# Autodesk Inventor assembly: CL3-100
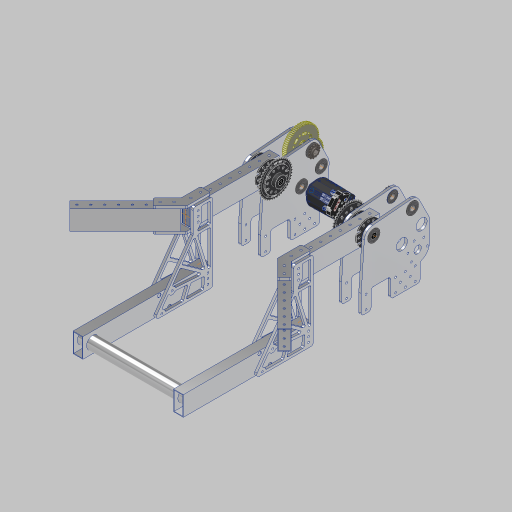
[picture p0: Inventor's stored thumbnail of the model, 512x512]
Saved by Autodesk Inventor 2023.5 (Build 275446000, 446)
## iProperties
Created: 2025-01-28
Part Number: CL3-100
Document SubType Name: Assembly
Designer: slick
Mass: 5966.39 g
Surface Area: 14199.1 cm^2
Volume: 2256.64 cm^3
Density: 2.64392 g/cm^3
Author: slick
## Documents named in this file (22)
- C:\Users\slick\OneDrive\Desktop\2025-ReefScape---CAD\Climber\CL3\CL3-100.iam
- C:\Users\slick\OneDrive\Desktop\2025-ReefScape---CAD\Climber\CL3\CL3-001.ipt
- C:\Users\slick\OneDrive\Desktop\2025-ReefScape---CAD\Climber\CL3\CL3-002.ipt
- C:\Users\slick\OneDrive\Desktop\2025-ReefScape---CAD\Climber\CL3\CL3-003.ipt
- C:\Users\slick\OneDrive\Desktop\2025-ReefScape---CAD\Climber\CL3\CL3-006.ipt
- C:\Users\slick\OneDrive\Desktop\2025-ReefScape---CAD\Field Items\Full Field\FE-2025\GE-25201.iam
- C:\Users\slick\OneDrive\Desktop\2025-ReefScape---CAD\Climber\CL3\CL3-009.ipt
- C:\Users\slick\OneDrive\Desktop\2025-ReefScape---CAD\Elevator\EL2\EL2-005.ipt
- C:\Users\slick\OneDrive\Desktop\2025-ReefScape---CAD\Climber\CL3\CL3-010.ipt
- C:\Users\slick\OneDrive\Desktop\2025-ReefScape---CAD\Climber\CL3\CL3-011.ipt
- C:\Users\slick\OneDrive\Desktop\2025-ReefScape---CAD\COMMON PARTS\HUBS\WCP-1388.ipt
- C:\Users\slick\OneDrive\Desktop\2025-ReefScape---CAD\COMMON PARTS\SPROCKETS\25\WCP-0967 42t 25_chain.ipt
- C:\Users\slick\OneDrive\Desktop\2025-ReefScape---CAD\Climber\CL3\CL3-013.ipt
- C:\Users\slick\OneDrive\Desktop\2025-ReefScape---CAD\Climber\CL3\CL3-014.ipt
- C:\Users\slick\OneDrive\Desktop\2025-ReefScape---CAD\Climber\CL3\CL3-015.ipt
- C:\Users\slick\OneDrive\Desktop\2025-ReefScape---CAD\COMMON PARTS\MOTORS\Kracken with Cover and Boards.iam
- C:\Users\slick\OneDrive\Desktop\2025-ReefScape---CAD\COMMON PARTS\GEARS\WCP-1006\WCP-1006.ipt
- C:\Users\slick\OneDrive\Desktop\2025-ReefScape---CAD\COMMON PARTS\GEARS\20dp .5 hex\72t_Aluminum_Spur_Gear_20_DP_1_2_Hex_Bore_217-3576.ipt
- C:\Users\slick\OneDrive\Desktop\2025-ReefScape---CAD\COMMON PARTS\GEARS\20dp .5 hex\66t_Aluminum_Spur_Gear_20_DP_1_2_Hex_Bore_VersaKeys_217-3223.ipt
- C:\Users\slick\OneDrive\Desktop\2025-ReefScape---CAD\COMMON PARTS\GEARS\20dp .5 hex\20t_Aluminum_Spur_Gear_20_DP_1_2_Hex_Bore_217-2702.ipt
- C:\Users\slick\OneDrive\Desktop\2025-ReefScape---CAD\COMMON PARTS\SPROCKETS\25\14t Steel Double Hub Sprocket (#25 Chain, 12 Hex Bore)\14t Steel Double Hub Sprocket (#25 Chain, 12 Hex Bore).ipt
- C:\Users\slick\OneDrive\Desktop\2025-ReefScape---CAD\COMMON PARTS\BEARINGS\13_75mm_1_2_ThunderHex_ID_x_1_125_OD_x_0_313_WD_Flanged_Bearing_217-4006_MIR.ipt
## Components (58 placed, 21 different names)
1. CL3-001:1 — Flush:24, Insert:5, Insert:6, Insert:7, Insert:11, Insert:12, Insert:13, Insert:14, Mate:43, Mate:44, Mate:51, Mate:52, Mate:53, Mate:54, Mate:55, Angle:4, Insert:43, Insert:44, Mate:90
2. CL3-002:1 — Flush:24, Insert:3, Insert:4, Insert:8
3. CL3-003:1 — Insert:26, Insert:27, Mate:56, Mate:57, Insert:48, Insert:49, Insert:50, Insert:51
4. CL3-001:2 — Insert:18, Insert:19, Insert:20, Insert:21, Insert:24, Insert:25, Insert:41, Mate:65, Insert:42, Mate:66, Mate:67
5. CL3-002:2 — Insert:22, Insert:23
6. CL3-003:2 — Mate:33, Mate:34, Insert:15, Insert:16, Insert:17, Insert:45, Insert:46, Insert:47
7. CL3-015:5 — Mate:41, Flush:31, Flush:32, Angle:4, Symmetry:2, Mate:76, Mate:85, Mate:87, Symmetry:4, Mate:93, Insert:61, Insert:62, Insert:63, Insert:64
8. CL3-015:4 — Mate:68, Flush:33, Symmetry:3, Mate:93, Symmetry:5, Insert:65, Insert:67, Flush:47
9. CL3-006:1 — Tangent:1, Mate:21, Mate:33, Mate:34, Mate:56, Mate:57
10. GE-25201:1 [sub-assembly] — Mate:20, Tangent:1, Mate:21
11. CL3-009:1 — Insert:3, Insert:4, Insert:5, Insert:6
12. CL3-009:2 — Insert:7, Insert:8
13. CL3-013:1 — Insert:43, Insert:44
14. CL3-010:1 — Insert:11, Insert:12, Flush:29
15. CL3-010:2 — Insert:13, Insert:14, Insert:16, Insert:17
16. EL2-005:3 — Insert:15, Insert:45
17. CL3-009:3 — Insert:18, Insert:19
18. CL3-009:4 — Insert:20, Insert:21, Insert:22, Insert:23
19. CL3-010:3 — Insert:25, Flush:29, Flush:30
20. CL3-010:4 — Insert:24, Insert:26, Insert:27, Flush:30
21. CL3-011:1 — Mate:55, Mate:81, Mate:96, Flush:48, Flush:49
22. CL3-015:2 — Mate:41, Flush:31, Flush:32, Symmetry:2, Flush:34, Flush:35, Mate:70, Insert:52, Mate:77, Mate:79, Mate:80, Mate:83, Symmetry:4, Insert:57, Insert:58, Insert:59, Insert:60
23. WCP-1388:1 — Mate:43, Mate:44, Mate:51
24. WCP-1388:2 — Mate:52, Mate:53, Mate:54
25. CL3-015:3 — Mate:68, Flush:33, Flush:34, Flush:35, Symmetry:3, Symmetry:5, Insert:66, Insert:68, Flush:47
26. CL3-011:2 — Mate:67, Mate:88, Mate:95, Flush:50, Flush:51
27. WCP-1388:3 — Insert:41, Mate:65
28. WCP-1388:4 — Insert:42, Mate:66
29. CL3-014:1 — Insert:46
30. CL3-014:2 — Insert:47
31. CL3-014:3 — Insert:50
32. CL3-014:4 — Insert:51
33. EL2-005:4 — Insert:48, Insert:49
34. Kracken with Cover and Boards:1 [sub-assembly] — Mate:70, Insert:52, Mate:72, Mate:73, Mate:79
35. WCP-1006:1 — Mate:72, Mate:73
36. 72t_Aluminum_Spur_Gear_20_DP_1_2_Hex_Bore_217-3576:1 — Mate:80, Mate:83, Mate:84
37. 20t_Aluminum_Spur_Gear_20_DP_1_2_Hex_Bore_217-2702:2 — Mate:84, Flush:39, Mate:85
38. 66t_Aluminum_Spur_Gear_20_DP_1_2_Hex_Bore_VersaKeys_217-3223:1 — Mate:76, Flush:39, Mate:86
39. 20t_Aluminum_Spur_Gear_20_DP_1_2_Hex_Bore_217-2702:1 — Mate:77, Flush:38, Mate:86
40. 66t_Aluminum_Spur_Gear_20_DP_1_2_Hex_Bore_VersaKeys_217-3223:2 — Flush:38
41. WCP-0967 42t 25_chain:3 — Insert:53, Insert:54, Flush:45
42. WCP-1388:5 — Insert:53, Insert:54, Mate:81, Flush:48
43. 14t Steel Double Hub Sprocket (#25 Chain, 12 Hex Bore):1 — Mate:87, Flush:45
44. WCP-0967 42t 25_chain:4 — Flush:46
45. WCP-1388:6 — Mate:88, Flush:50
46. 13_75mm_1_2_ThunderHex_ID_x_1_125_OD_x_0_313_WD_Flanged_Bearing_217-4006_MIR:1 — Insert:68
47. 13_75mm_1_2_ThunderHex_ID_x_1_125_OD_x_0_313_WD_Flanged_Bearing_217-4006_MIR:2 — Insert:67, Mate:95, Flush:51
48. 13_75mm_1_2_ThunderHex_ID_x_1_125_OD_x_0_313_WD_Flanged_Bearing_217-4006_MIR:3 — Insert:65
49. 13_75mm_1_2_ThunderHex_ID_x_1_125_OD_x_0_313_WD_Flanged_Bearing_217-4006_MIR:4 — Insert:66, Mate:94
50. 13_75mm_1_2_ThunderHex_ID_x_1_125_OD_x_0_313_WD_Flanged_Bearing_217-4006_MIR:5 — Insert:58
51. 13_75mm_1_2_ThunderHex_ID_x_1_125_OD_x_0_313_WD_Flanged_Bearing_217-4006_MIR:6 — Insert:57
52. 13_75mm_1_2_ThunderHex_ID_x_1_125_OD_x_0_313_WD_Flanged_Bearing_217-4006_MIR:7 — Insert:61
53. 13_75mm_1_2_ThunderHex_ID_x_1_125_OD_x_0_313_WD_Flanged_Bearing_217-4006_MIR:8 — Insert:59
54. 13_75mm_1_2_ThunderHex_ID_x_1_125_OD_x_0_313_WD_Flanged_Bearing_217-4006_MIR:9 — Insert:62
55. 13_75mm_1_2_ThunderHex_ID_x_1_125_OD_x_0_313_WD_Flanged_Bearing_217-4006_MIR:10 — Insert:60, Mate:96
56. 13_75mm_1_2_ThunderHex_ID_x_1_125_OD_x_0_313_WD_Flanged_Bearing_217-4006_MIR:11 — Insert:64, Flush:49
57. 13_75mm_1_2_ThunderHex_ID_x_1_125_OD_x_0_313_WD_Flanged_Bearing_217-4006_MIR:12 — Insert:63
58. 14t Steel Double Hub Sprocket (#25 Chain, 12 Hex Bore):2 — Mate:94, Flush:46
## Relationships (114: Insert 51, Mate 40, Flush 17, Symmetry 4, Tangent 1, Angle 1)
- Mate:20: GE-25201:1
- Tangent:1: CL3-006:1 ↔ GE-25201:1
- Mate:21 (-76.2 mm): CL3-006:1 ↔ GE-25201:1
- Flush:24: CL3-001:1 ↔ CL3-002:1
- Insert:3: CL3-002:1 ↔ CL3-009:1
- Insert:4: CL3-002:1 ↔ CL3-009:1
- Insert:5: CL3-001:1 ↔ CL3-009:1
- Insert:6: CL3-001:1 ↔ CL3-009:1
- Insert:7: CL3-001:1 ↔ CL3-009:2
- Insert:8: CL3-002:1 ↔ CL3-009:2
- Mate:33: CL3-003:2 ↔ CL3-006:1
- Mate:34: CL3-003:2 ↔ CL3-006:1
- Insert:11: CL3-001:1 ↔ CL3-010:1
- Insert:12: CL3-001:1 ↔ CL3-010:1
- Insert:13: CL3-001:1 ↔ CL3-010:2
- Insert:14: CL3-001:1 ↔ CL3-010:2
- Insert:15: CL3-003:2 ↔ EL2-005:3
- Insert:16: CL3-003:2 ↔ CL3-010:2
- Insert:17: CL3-003:2 ↔ CL3-010:2
- Insert:18: CL3-001:2 ↔ CL3-009:3
- Insert:19: CL3-001:2 ↔ CL3-009:3
- Insert:20: CL3-001:2 ↔ CL3-009:4
- Insert:21: CL3-001:2 ↔ CL3-009:4
- Insert:22: CL3-002:2 ↔ CL3-009:4
- Insert:23: CL3-002:2 ↔ CL3-009:4
- Insert:24: CL3-001:2 ↔ CL3-010:4
- Insert:25: CL3-001:2 ↔ CL3-010:3
- Flush:29: CL3-010:1 ↔ CL3-010:3
- Insert:26: CL3-003:1 ↔ CL3-010:4
- Insert:27: CL3-003:1 ↔ CL3-010:4
- Flush:30: CL3-010:3 ↔ CL3-010:4
- Mate:41 (44.45 mm): CL3-015:5 ↔ CL3-015:2
- Flush:31: CL3-015:5 ↔ CL3-015:2
- Flush:32: CL3-015:5 ↔ CL3-015:2
- Mate:43: CL3-001:1 ↔ WCP-1388:1
- Mate:44: CL3-001:1 ↔ WCP-1388:1
- Mate:51: CL3-001:1 ↔ WCP-1388:1
- Mate:52: CL3-001:1 ↔ WCP-1388:2
- Mate:53: CL3-001:1 ↔ WCP-1388:2
- Mate:54: CL3-001:1 ↔ WCP-1388:2
- Mate:55: CL3-001:1 ↔ CL3-011:1
- Angle:4 (270 deg): CL3-001:1 ↔ CL3-015:5
- Mate:56: CL3-003:1 ↔ CL3-006:1
- Mate:57: CL3-003:1 ↔ CL3-006:1
- Symmetry:2: CL3-015:5 ↔ CL3-015:2
- Mate:59
- Insert:41: CL3-001:2 ↔ WCP-1388:3
- Mate:65: CL3-001:2 ↔ WCP-1388:3
- Insert:42: CL3-001:2 ↔ WCP-1388:4
- Mate:66: CL3-001:2 ↔ WCP-1388:4
- Mate:67: CL3-001:2 ↔ CL3-011:2
- Mate:68 (44.45 mm): CL3-015:4 ↔ CL3-015:3
- Flush:33: CL3-015:4 ↔ CL3-015:3
- Flush:34: CL3-015:2 ↔ CL3-015:3
- Flush:35: CL3-015:2 ↔ CL3-015:3
- Symmetry:3: CL3-015:4 ↔ CL3-015:3
- Mate:69
- Insert:43: CL3-001:1 ↔ CL3-013:1
- Insert:44: CL3-001:1 ↔ CL3-013:1
- Insert:45: CL3-003:2 ↔ EL2-005:3
- Insert:46: CL3-003:2 ↔ CL3-014:1
- Insert:47: CL3-003:2 ↔ CL3-014:2
- Insert:48: CL3-003:1 ↔ EL2-005:4
- Insert:49: CL3-003:1 ↔ EL2-005:4
- Insert:50: CL3-003:1 ↔ CL3-014:3
- Insert:51: CL3-003:1 ↔ CL3-014:4
- Mate:70: CL3-015:2 ↔ Kracken with Cover and Boards:1
- Insert:52: CL3-015:2 ↔ Kracken with Cover and Boards:1
- Mate:72: Kracken with Cover and Boards:1 ↔ WCP-1006:1
- Mate:73 (3.175 mm): Kracken with Cover and Boards:1 ↔ WCP-1006:1
- Mate:76: CL3-015:5 ↔ 66t_Aluminum_Spur_Gear_20_DP_1_2_Hex_Bore_VersaKeys_217-3223:1
- Mate:77: CL3-015:2 ↔ 20t_Aluminum_Spur_Gear_20_DP_1_2_Hex_Bore_217-2702:1
- [Mate]: CL3-015:2 ↔ 66t_Aluminum_Spur_Gear_20_DP_1_2_Hex_Bore_VersaKeys_217-3223:2
- Mate:79: CL3-015:2 ↔ Kracken with Cover and Boards:1
- Mate:80: CL3-015:2 ↔ 72t_Aluminum_Spur_Gear_20_DP_1_2_Hex_Bore_217-3576:1
- Flush:38: 20t_Aluminum_Spur_Gear_20_DP_1_2_Hex_Bore_217-2702:1 ↔ 66t_Aluminum_Spur_Gear_20_DP_1_2_Hex_Bore_VersaKeys_217-3223:2
- Insert:53: WCP-0967 42t 25_chain:3 ↔ WCP-1388:5
- Insert:54: WCP-0967 42t 25_chain:3 ↔ WCP-1388:5
- Mate:81: CL3-011:1 ↔ WCP-1388:5
- Mate:83 (3.175 mm): CL3-015:2 ↔ 72t_Aluminum_Spur_Gear_20_DP_1_2_Hex_Bore_217-3576:1
- Mate:84: 72t_Aluminum_Spur_Gear_20_DP_1_2_Hex_Bore_217-3576:1 ↔ 20t_Aluminum_Spur_Gear_20_DP_1_2_Hex_Bore_217-2702:2
- Flush:39: 20t_Aluminum_Spur_Gear_20_DP_1_2_Hex_Bore_217-2702:2 ↔ 66t_Aluminum_Spur_Gear_20_DP_1_2_Hex_Bore_VersaKeys_217-3223:1
- Mate:85 (3.175 mm): CL3-015:5 ↔ 20t_Aluminum_Spur_Gear_20_DP_1_2_Hex_Bore_217-2702:2
- Mate:86: 66t_Aluminum_Spur_Gear_20_DP_1_2_Hex_Bore_VersaKeys_217-3223:1 ↔ 20t_Aluminum_Spur_Gear_20_DP_1_2_Hex_Bore_217-2702:1
- Mate:87: CL3-015:5 ↔ 14t Steel Double Hub Sprocket (#25 Chain, 12 Hex Bore):1
- [Insert]: WCP-0967 42t 25_chain:4 ↔ WCP-1388:6
- [Insert]: WCP-0967 42t 25_chain:4 ↔ WCP-1388:6
- Mate:88: CL3-011:2 ↔ WCP-1388:6
- Symmetry:4: CL3-015:5 ↔ CL3-015:2
- Mate:90: CL3-001:1
- Mate:93 (304.8 mm): CL3-015:5 ↔ CL3-015:4
- Symmetry:5: CL3-015:4 ↔ CL3-015:3
- Flush:45: WCP-0967 42t 25_chain:3 ↔ 14t Steel Double Hub Sprocket (#25 Chain, 12 Hex Bore):1
- Insert:57: CL3-015:2 ↔ 13_75mm_1_2_ThunderHex_ID_x_1_125_OD_x_0_313_WD_Flanged_Bearing_217-4006_MIR:6
- Insert:58: CL3-015:2 ↔ 13_75mm_1_2_ThunderHex_ID_x_1_125_OD_x_0_313_WD_Flanged_Bearing_217-4006_MIR:5
- Insert:59: CL3-015:2 ↔ 13_75mm_1_2_ThunderHex_ID_x_1_125_OD_x_0_313_WD_Flanged_Bearing_217-4006_MIR:8
- Insert:60: CL3-015:2 ↔ 13_75mm_1_2_ThunderHex_ID_x_1_125_OD_x_0_313_WD_Flanged_Bearing_217-4006_MIR:10
- Insert:61: CL3-015:5 ↔ 13_75mm_1_2_ThunderHex_ID_x_1_125_OD_x_0_313_WD_Flanged_Bearing_217-4006_MIR:7
- Insert:62: CL3-015:5 ↔ 13_75mm_1_2_ThunderHex_ID_x_1_125_OD_x_0_313_WD_Flanged_Bearing_217-4006_MIR:9
- Insert:63: CL3-015:5 ↔ 13_75mm_1_2_ThunderHex_ID_x_1_125_OD_x_0_313_WD_Flanged_Bearing_217-4006_MIR:12
- Insert:64: CL3-015:5 ↔ 13_75mm_1_2_ThunderHex_ID_x_1_125_OD_x_0_313_WD_Flanged_Bearing_217-4006_MIR:11
- Insert:65: CL3-015:4 ↔ 13_75mm_1_2_ThunderHex_ID_x_1_125_OD_x_0_313_WD_Flanged_Bearing_217-4006_MIR:3
- Insert:66: CL3-015:3 ↔ 13_75mm_1_2_ThunderHex_ID_x_1_125_OD_x_0_313_WD_Flanged_Bearing_217-4006_MIR:4
- Insert:67: CL3-015:4 ↔ 13_75mm_1_2_ThunderHex_ID_x_1_125_OD_x_0_313_WD_Flanged_Bearing_217-4006_MIR:2
- Insert:68: CL3-015:3 ↔ 13_75mm_1_2_ThunderHex_ID_x_1_125_OD_x_0_313_WD_Flanged_Bearing_217-4006_MIR:1
- Mate:94: 13_75mm_1_2_ThunderHex_ID_x_1_125_OD_x_0_313_WD_Flanged_Bearing_217-4006_MIR:4 ↔ 14t Steel Double Hub Sprocket (#25 Chain, 12 Hex Bore):2
- Flush:46: WCP-0967 42t 25_chain:4 ↔ 14t Steel Double Hub Sprocket (#25 Chain, 12 Hex Bore):2
- Mate:95: CL3-011:2 ↔ 13_75mm_1_2_ThunderHex_ID_x_1_125_OD_x_0_313_WD_Flanged_Bearing_217-4006_MIR:2
- Flush:47: CL3-015:4 ↔ CL3-015:3
- Mate:96: CL3-011:1 ↔ 13_75mm_1_2_ThunderHex_ID_x_1_125_OD_x_0_313_WD_Flanged_Bearing_217-4006_MIR:10
- Flush:48: CL3-011:1 ↔ WCP-1388:5
- Flush:49: CL3-011:1 ↔ 13_75mm_1_2_ThunderHex_ID_x_1_125_OD_x_0_313_WD_Flanged_Bearing_217-4006_MIR:11
- Flush:50: CL3-011:2 ↔ WCP-1388:6
- Flush:51: CL3-011:2 ↔ 13_75mm_1_2_ThunderHex_ID_x_1_125_OD_x_0_313_WD_Flanged_Bearing_217-4006_MIR:2
## Named parameters: d266_d254 = 0 mm, d267_d255 = 0 mm
